# Autodesk Inventor assembly: ForeArmAssembly
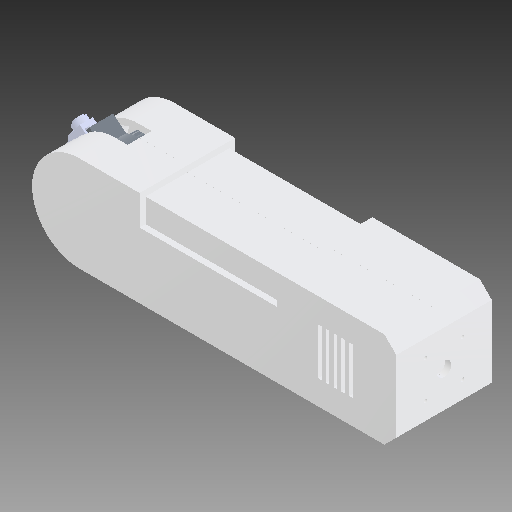
[picture p0: Inventor's stored thumbnail of the model, 512x512]
Saved by Autodesk Inventor 2017 SP1 (Build 210196100, 196)
## iProperties
Created: 2017-06-16
Part Number: ForeArmAssembly
Document SubType Name: Assembly
Designer: Zach
Author: Zach
## Documents named in this file (11)
- C:\Users\Zach\Documents\GitHub\cr-laundry-robot\src\Body\Arm Assembly\Fore Arm Assembly\ForeArmAssembly.iam
- C:\Users\Zach\Documents\GitHub\cr-laundry-robot\src\Body\Arm Assembly\Fore Arm Assembly\FA001.ipt
- C:\Users\Zach\Documents\GitHub\cr-laundry-robot\src\Body\Arm Assembly\Fore Arm Assembly\FA002.ipt
- C:\Users\Zach\Documents\GitHub\cr-laundry-robot\src\Body\Arm Assembly\Fore Arm Assembly\FA003.ipt
- C:\Users\Zach\Documents\GitHub\cr-laundry-robot\src\Body\Arm Assembly\Fore Arm Assembly\FA004.ipt
- C:\Users\Zach\Documents\GitHub\cr-laundry-robot\src\Body\Arm Assembly\Fore Arm Assembly\FA005.ipt
- C:\Users\Zach\Documents\GitHub\cr-laundry-robot\lib\Stepper Motor - NEMA 17\NEMA17.ipt
- C:\Users\Zach\Documents\GitHub\cr-laundry-robot\src\Body\Arm Assembly\Fore Arm Assembly\FA006.ipt
- C:\Users\Zach\Documents\GitHub\cr-laundry-robot\src\Body\Arm Assembly\Fore Arm Assembly\FA007.ipt
- C:\Users\Zach\Documents\GitHub\cr-laundry-robot\src\Body\Arm Assembly\Fore Arm Assembly\FA008.ipt
- C:\Users\Zach\Documents\GitHub\cr-laundry-robot\lib\Futaba S3114\FutabaS3114.ipt
## Components (11 placed, 10 different names)
1. FA001:1 — Mate:3, Mate:4, Mate:12, Mate:13, Mate:14, Mate:15, Mate:16
2. FA002:1 — Mate:15, Mate:16
3. FA003:1 — Mate:3, Mate:4, Mate:10, Mate:11, Mate:17, Mate:18, Mate:19, Mate:20, Mate:21, Mate:23
4. FA004:1
5. FA005:1 — Mate:10, Mate:11, Mate:24, Mate:25
6. NEMA17:1 — Mate:12, Mate:13, Mate:14
7. NEMA17:2 — Mate:17, Mate:18, Mate:19, Mate:22
8. FA006:1 — Mate:20, Mate:21
9. FA007:1 — Mate:22, Mate:23
10. FA008:1 — Mate:24, Mate:25, Mate:26, Mate:27
11. FutabaS3114:1 — Mate:26, Mate:27
## Relationships (20: Mate 20)
- Mate:3: FA001:1 ↔ FA003:1
- Mate:4: FA001:1 ↔ FA003:1
- Mate:10: FA003:1 ↔ FA005:1
- Mate:11: FA003:1 ↔ FA005:1
- Mate:12: FA001:1 ↔ NEMA17:1
- Mate:13: FA001:1 ↔ NEMA17:1
- Mate:14: FA001:1 ↔ NEMA17:1
- Mate:15: FA001:1 ↔ FA002:1
- Mate:16: FA001:1 ↔ FA002:1
- Mate:17: FA003:1 ↔ NEMA17:2
- Mate:18: FA003:1 ↔ NEMA17:2
- Mate:19: FA003:1 ↔ NEMA17:2
- Mate:20: FA003:1 ↔ FA006:1
- Mate:21: FA003:1 ↔ FA006:1
- Mate:22: NEMA17:2 ↔ FA007:1
- Mate:23: FA003:1 ↔ FA007:1
- Mate:24: FA005:1 ↔ FA008:1
- Mate:25: FA005:1 ↔ FA008:1
- Mate:26: FA008:1 ↔ FutabaS3114:1
- Mate:27: FA008:1 ↔ FutabaS3114:1
